# Autodesk Inventor assembly: CE-8.2.2
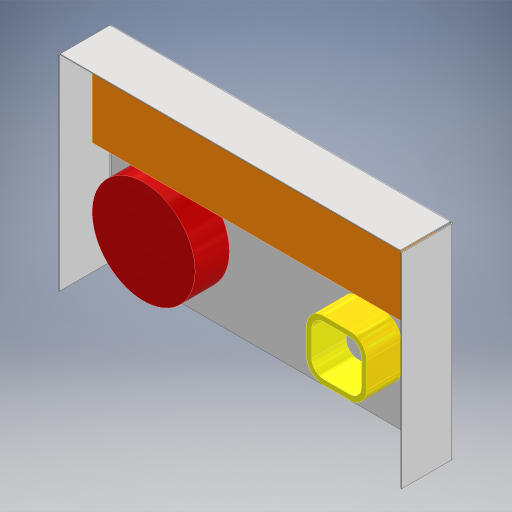
[picture p0: Inventor's stored thumbnail of the model, 512x512]
Saved by Autodesk Inventor 2024 (Build 280153000, 153)
## iProperties
Created: 2024-03-07
Part Number: CE-8.2.2
Document SubType Name: Assembly
Designer: Alex
Author: Alex
## Documents named in this file (5)
- C:\Shared\alex-bartella-schoolwork\4z03\Week 8\CE-8.2.2.iam
- C:\Shared\alex-bartella-schoolwork\4z03\Week 8\CE-8.2.2-01-001.ipt
- C:\Shared\alex-bartella-schoolwork\4z03\Week 8\CE-8.2.2-01-002.ipt
- C:\Shared\alex-bartella-schoolwork\4z03\Week 8\CE-8.2.2-01-003.ipt
- C:\Shared\alex-bartella-schoolwork\4z03\Week 8\CE-8.2.2-01-004.ipt
## Components (4 placed, 4 different names)
1. CE-8.2.2-01-001:1 — Flush:1
2. CE-8.2.2-01-002:1 — Flush:2
3. CE-8.2.2-01-003:1 — Flush:3
4. CE-8.2.2-01-004:1 — Flush:4
## Relationships (4: Flush 4)
- Flush:1: CE-8.2.2-01-001:1
- Flush:2: CE-8.2.2-01-002:1
- Flush:3: CE-8.2.2-01-003:1
- Flush:4: CE-8.2.2-01-004:1
